# Autodesk Inventor assembly: Mechanism Platform
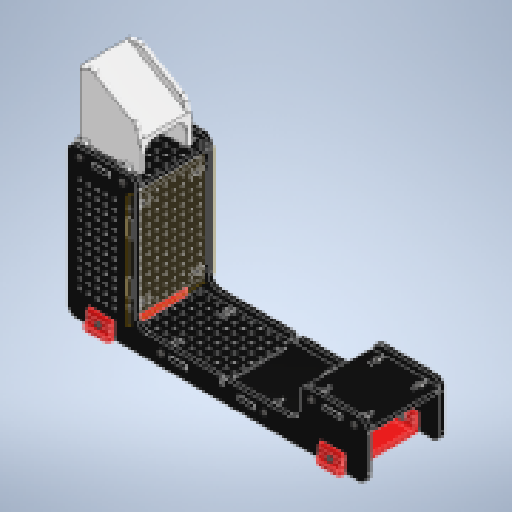
[picture p0: Inventor's stored thumbnail of the model, 512x512]
Saved by Autodesk Inventor 2025.1 (Build 291241000, 241)
## iProperties
Manager: Yassa Basem
Company: ENG 1P13
Created: 2024-06-07
Part Number: Mechanism Platform
Document SubType Name: Assembly
Designer: Alex Forbes
Checked By: Yassa Basem
Engineer: Alex Forbes
Author: A 1P13 IAI
Title: Mechanism Platform
## Documents named in this file (11)
- C:\Users\hanna\OneDrive - McMaster University\Documents\ENG 1P13A\Project 1\New folder (1)\Mechanism Platform.iam
- C:\Users\hanna\OneDrive - McMaster University\Documents\ENG 1P13A\Project 1\New folder (1)\Mounting Base Middle.ipt
- C:\Users\hanna\OneDrive - McMaster University\Documents\ENG 1P13A\Project 1\New folder (1)\Mounting Base Side.ipt
- C:\Users\hanna\OneDrive - McMaster University\Documents\ENG 1P13A\Project 1\New folder (1)\ANSI B 18.2.4.1 M - M4 x 0.7Style 1.ipt
- C:\Users\hanna\OneDrive - McMaster University\Documents\ENG 1P13A\Project 1\New folder (1)\Mounting Base Bottom.ipt
- C:\Users\hanna\OneDrive - McMaster University\Documents\ENG 1P13A\Project 1\New folder (1)\ANSI B18.6.7M - M4x0.7 x 20(4).ipt
- C:\Users\hanna\OneDrive - McMaster University\Documents\ENG 1P13A\Project 1\New folder (1)\Mounting Feet.ipt
- C:\Users\hanna\OneDrive - McMaster University\Documents\ENG 1P13A\Project 1\New folder (1)\Mounting Side Wall.ipt
- C:\Users\hanna\OneDrive - McMaster University\Documents\ENG 1P13A\Project 1\New folder (1)\Mounting Base Top.ipt
- C:\Users\hanna\OneDrive - McMaster University\Documents\ENG 1P13A\Project 1\New folder (1)\Top Ramp.ipt
- C:\Users\hanna\OneDrive - McMaster University\Documents\ENG 1P13A\Project 1\New folder (1)\M4 x 20mm Machine Screw.ipt
## Components (53 placed, 10 different names)
1. Top Ramp:1 — Insert:3, Insert:4, Insert:6, Insert:7, Insert:8, Insert:9, Insert:10, Insert:11, Angle:8, Angle:9, Angle:10, Angle:11
2. M4 x 20mm Machine Screw:1 — Insert:3, Angle:9
3. M4 x 20mm Machine Screw:2 — Insert:7, Angle:8
4. M4 x 20mm Machine Screw:3 — Insert:4, Angle:10
5. M4 x 20mm Machine Screw:4 — Insert:6, Angle:11
6. Mounting Side Wall:1 — Insert:1, Angle:1, Insert:2, Mate:1, Mate:2, Mate:3, Mate:4, Flush:1, Flush:2, Mate:5, Angle:3, Mate:6, Mate:7, Mate:8, Mate:9, Mate:50, Mate:51, Mate:52, Mate:53, Mate:109, Mate:110, Mate:111, Mate:129, Mate:130, Mate:131, Mate:133, Mate:134, Mate:135, Mate:145, Mate:146, Mate:147, Mate:149, Mate:150, Mate:151, Mate:157, Mate:158, Mate:159, Mate:169, Mate:170, Mate:171, Mate:173, Mate:174, Mate:175
7. Mounting Side Wall:2 — Mate:4, Flush:1, Flush:2, Mate:117, Mate:118, Mate:119, Mate:121, Mate:122, Mate:123, Mate:125, Mate:126, Mate:127, Mate:137, Mate:138, Mate:139, Mate:141, Mate:142, Mate:143, Mate:153, Mate:154, Mate:155, Mate:161, Mate:162, Mate:163, Mate:165, Mate:166, Mate:167
8. Mounting Base Top:1 — Mate:1, Mate:8, Mate:9, Mate:112, Mate:120, Mate:124, Mate:176, Angle:6, Angle:7, Insert:8, Insert:9, Insert:10, Insert:11
9. Mounting Base Middle:1 — Mate:2, Mate:52, Mate:53, Mate:144, Mate:148, Mate:152, Mate:156
10. Mounting Base Bottom:1 — Mate:3, Mate:50, Mate:51, Mate:160, Mate:164, Mate:168, Mate:172, Angle:4, Angle:5
11. Mounting Base Side:1 — Mate:5, Angle:3, Mate:6, Mate:7, Mate:128, Mate:132, Mate:136, Mate:140, Flush:3
12. Mounting Feet:1 — Insert:1, Angle:1, Angle:2, Mate:177, Mate:178, Mate:179, Mate:180, Mate:181, Mate:182, Mate:183, Mate:184
13. Mounting Feet:2 — Insert:2, Angle:2, Mate:185, Mate:186, Mate:187, Mate:188, Mate:189, Mate:190, Mate:191, Mate:192
14. Cross Recessed Pan Head Machine Screw - Type I - Metric M4x0.7 x 20:1 — Mate:173, Mate:174
15. Hex Nut Metric M4 x 0.7:1 — Mate:175, Mate:176
16. Cross Recessed Pan Head Machine Screw - Type I - Metric M4x0.7 x 20:7 — Mate:129, Mate:130
17. Hex Nut Metric M4 x 0.7:3 — Mate:131, Mate:132
18. Cross Recessed Pan Head Machine Screw - Type I - Metric M4x0.7 x 20:8 — Mate:133, Mate:134
19. Hex Nut Metric M4 x 0.7:5 — Mate:135, Mate:136
20. Cross Recessed Pan Head Machine Screw - Type I - Metric M4x0.7 x 20:5 — Mate:121, Mate:122
21. Hex Nut Metric M4 x 0.7:6 — Mate:123, Mate:124
22. Cross Recessed Pan Head Machine Screw - Type I - Metric M4x0.7 x 20:4 — Mate:117, Mate:118
23. Hex Nut Metric M4 x 0.7:7 — Mate:119, Mate:120
24. Cross Recessed Pan Head Machine Screw - Type I - Metric M4x0.7 x 20:6 — Mate:125, Mate:126
25. Hex Nut Metric M4 x 0.7:8 — Mate:127, Mate:128
26. Cross Recessed Pan Head Machine Screw - Type I - Metric M4x0.7 x 20:3 — Mate:137, Mate:138
27. Hex Nut Metric M4 x 0.7:10 — Mate:139, Mate:140
28. Cross Recessed Pan Head Machine Screw - Type I - Metric M4x0.7 x 20:10 — Mate:145, Mate:146
29. Hex Nut Metric M4 x 0.7:11 — Mate:147, Mate:148
30. Cross Recessed Pan Head Machine Screw - Type I - Metric M4x0.7 x 20:11 — Mate:149, Mate:150
31. Hex Nut Metric M4 x 0.7:13 — Mate:151, Mate:152
32. Cross Recessed Pan Head Machine Screw - Type I - Metric M4x0.7 x 20:9 — Mate:141, Mate:142
33. Hex Nut Metric M4 x 0.7:14 — Mate:143, Mate:144
34. Cross Recessed Pan Head Machine Screw - Type I - Metric M4x0.7 x 20:12 — Mate:153, Mate:154
35. Hex Nut Metric M4 x 0.7:16 — Mate:155, Mate:156
36. Cross Recessed Pan Head Machine Screw - Type I - Metric M4x0.7 x 20:13 — Mate:157, Mate:158
37. Hex Nut Metric M4 x 0.7:17 — Mate:159, Mate:160
38. Cross Recessed Pan Head Machine Screw - Type I - Metric M4x0.7 x 20:16 — Mate:169, Mate:170
39. Hex Nut Metric M4 x 0.7:18 — Mate:171, Mate:172
40. Cross Recessed Pan Head Machine Screw - Type I - Metric M4x0.7 x 20:14 — Mate:161, Mate:162
41. Hex Nut Metric M4 x 0.7:19 — Mate:163, Mate:164
42. Cross Recessed Pan Head Machine Screw - Type I - Metric M4x0.7 x 20:15 — Mate:165, Mate:166
43. Hex Nut Metric M4 x 0.7:20 — Mate:167, Mate:168
44. Cross Recessed Pan Head Machine Screw - Type I - Metric M4x0.7 x 20:2 — Mate:109, Mate:110
45. Hex Nut Metric M4 x 0.7:21 — Mate:111, Mate:112
46. Cross Recessed Pan Head Machine Screw - Type I - Metric M4x0.7 x 20:17 — Mate:177, Mate:178
47. Hex Nut Metric M4 x 0.7:22 — Mate:179, Mate:180, Angle:6
48. Cross Recessed Pan Head Machine Screw - Type I - Metric M4x0.7 x 20:18 — Mate:181, Mate:182
49. Hex Nut Metric M4 x 0.7:23 — Mate:183, Mate:184, Angle:7
50. Cross Recessed Pan Head Machine Screw - Type I - Metric M4x0.7 x 20:19 — Mate:185, Mate:186
51. Hex Nut Metric M4 x 0.7:24 — Mate:187, Mate:188, Angle:5
52. Cross Recessed Pan Head Machine Screw - Type I - Metric M4x0.7 x 20:20 — Mate:189, Mate:190
53. Hex Nut Metric M4 x 0.7:25 — Mate:191, Mate:192, Angle:4
## Relationships (117: Mate 93, Angle 11, Insert 10, Flush 3)
- Insert:1: Mounting Side Wall:1 ↔ Mounting Feet:1
- Angle:1 (0 deg): Mounting Side Wall:1 ↔ Mounting Feet:1
- Insert:2: Mounting Side Wall:1 ↔ Mounting Feet:2
- Angle:2 (0 deg): Mounting Feet:1 ↔ Mounting Feet:2
- Mate:1: Mounting Side Wall:1 ↔ Mounting Base Top:1
- Mate:2: Mounting Side Wall:1 ↔ Mounting Base Middle:1
- Mate:3: Mounting Side Wall:1 ↔ Mounting Base Bottom:1
- Mate:4 (102.3 mm): Mounting Side Wall:1 ↔ Mounting Side Wall:2
- Flush:1: Mounting Side Wall:1 ↔ Mounting Side Wall:2
- Flush:2: Mounting Side Wall:1 ↔ Mounting Side Wall:2
- Mate:5: Mounting Side Wall:1 ↔ Mounting Base Side:1
- Angle:3 (0 deg): Mounting Side Wall:1 ↔ Mounting Base Side:1
- Mate:6: Mounting Side Wall:1 ↔ Mounting Base Side:1
- Mate:7: Mounting Side Wall:1 ↔ Mounting Base Side:1
- Mate:8: Mounting Side Wall:1 ↔ Mounting Base Top:1
- Mate:9: Mounting Side Wall:1 ↔ Mounting Base Top:1
- Mate:50: Mounting Side Wall:1 ↔ Mounting Base Bottom:1
- Mate:51: Mounting Side Wall:1 ↔ Mounting Base Bottom:1
- Mate:52: Mounting Side Wall:1 ↔ Mounting Base Middle:1
- Mate:53: Mounting Side Wall:1 ↔ Mounting Base Middle:1
- Mate:109: Mounting Side Wall:1 ↔ Cross Recessed Pan Head Machine Screw - Type I - Metric M4x0.7 x 20:2
- Mate:110: Mounting Side Wall:1 ↔ Cross Recessed Pan Head Machine Screw - Type I - Metric M4x0.7 x 20:2
- Mate:111: Mounting Side Wall:1 ↔ Hex Nut Metric M4 x 0.7:21
- Mate:112: Mounting Base Top:1 ↔ Hex Nut Metric M4 x 0.7:21
- Mate:117: Mounting Side Wall:2 ↔ Cross Recessed Pan Head Machine Screw - Type I - Metric M4x0.7 x 20:4
- Mate:118: Mounting Side Wall:2 ↔ Cross Recessed Pan Head Machine Screw - Type I - Metric M4x0.7 x 20:4
- Mate:119: Mounting Side Wall:2 ↔ Hex Nut Metric M4 x 0.7:7
- Mate:120: Mounting Base Top:1 ↔ Hex Nut Metric M4 x 0.7:7
- Mate:121: Mounting Side Wall:2 ↔ Cross Recessed Pan Head Machine Screw - Type I - Metric M4x0.7 x 20:5
- Mate:122: Mounting Side Wall:2 ↔ Cross Recessed Pan Head Machine Screw - Type I - Metric M4x0.7 x 20:5
- Mate:123: Mounting Side Wall:2 ↔ Hex Nut Metric M4 x 0.7:6
- Mate:124: Mounting Base Top:1 ↔ Hex Nut Metric M4 x 0.7:6
- Mate:125: Mounting Side Wall:2 ↔ Cross Recessed Pan Head Machine Screw - Type I - Metric M4x0.7 x 20:6
- Mate:126: Mounting Side Wall:2 ↔ Cross Recessed Pan Head Machine Screw - Type I - Metric M4x0.7 x 20:6
- Mate:127: Mounting Side Wall:2 ↔ Hex Nut Metric M4 x 0.7:8
- Mate:128: Mounting Base Side:1 ↔ Hex Nut Metric M4 x 0.7:8
- Mate:129: Mounting Side Wall:1 ↔ Cross Recessed Pan Head Machine Screw - Type I - Metric M4x0.7 x 20:7
- Mate:130: Mounting Side Wall:1 ↔ Cross Recessed Pan Head Machine Screw - Type I - Metric M4x0.7 x 20:7
- Mate:131: Mounting Side Wall:1 ↔ Hex Nut Metric M4 x 0.7:3
- Mate:132: Mounting Base Side:1 ↔ Hex Nut Metric M4 x 0.7:3
- Mate:133: Mounting Side Wall:1 ↔ Cross Recessed Pan Head Machine Screw - Type I - Metric M4x0.7 x 20:8
- Mate:134: Mounting Side Wall:1 ↔ Cross Recessed Pan Head Machine Screw - Type I - Metric M4x0.7 x 20:8
- Mate:135: Mounting Side Wall:1 ↔ Hex Nut Metric M4 x 0.7:5
- Mate:136: Mounting Base Side:1 ↔ Hex Nut Metric M4 x 0.7:5
- Mate:137: Mounting Side Wall:2 ↔ Cross Recessed Pan Head Machine Screw - Type I - Metric M4x0.7 x 20:3
- Mate:138: Mounting Side Wall:2 ↔ Cross Recessed Pan Head Machine Screw - Type I - Metric M4x0.7 x 20:3
- Mate:139: Mounting Side Wall:2 ↔ Hex Nut Metric M4 x 0.7:10
- Mate:140: Mounting Base Side:1 ↔ Hex Nut Metric M4 x 0.7:10
- Mate:141: Mounting Side Wall:2 ↔ Cross Recessed Pan Head Machine Screw - Type I - Metric M4x0.7 x 20:9
- Mate:142: Mounting Side Wall:2 ↔ Cross Recessed Pan Head Machine Screw - Type I - Metric M4x0.7 x 20:9
- Mate:143: Mounting Side Wall:2 ↔ Hex Nut Metric M4 x 0.7:14
- Mate:144: Mounting Base Middle:1 ↔ Hex Nut Metric M4 x 0.7:14
- Mate:145: Mounting Side Wall:1 ↔ Cross Recessed Pan Head Machine Screw - Type I - Metric M4x0.7 x 20:10
- Mate:146: Mounting Side Wall:1 ↔ Cross Recessed Pan Head Machine Screw - Type I - Metric M4x0.7 x 20:10
- Mate:147: Mounting Side Wall:1 ↔ Hex Nut Metric M4 x 0.7:11
- Mate:148: Mounting Base Middle:1 ↔ Hex Nut Metric M4 x 0.7:11
- Mate:149: Mounting Side Wall:1 ↔ Cross Recessed Pan Head Machine Screw - Type I - Metric M4x0.7 x 20:11
- Mate:150: Mounting Side Wall:1 ↔ Cross Recessed Pan Head Machine Screw - Type I - Metric M4x0.7 x 20:11
- Mate:151: Mounting Side Wall:1 ↔ Hex Nut Metric M4 x 0.7:13
- Mate:152: Mounting Base Middle:1 ↔ Hex Nut Metric M4 x 0.7:13
- Mate:153: Mounting Side Wall:2 ↔ Cross Recessed Pan Head Machine Screw - Type I - Metric M4x0.7 x 20:12
- Mate:154: Mounting Side Wall:2 ↔ Cross Recessed Pan Head Machine Screw - Type I - Metric M4x0.7 x 20:12
- Mate:155: Mounting Side Wall:2 ↔ Hex Nut Metric M4 x 0.7:16
- Mate:156: Mounting Base Middle:1 ↔ Hex Nut Metric M4 x 0.7:16
- Mate:157: Mounting Side Wall:1 ↔ Cross Recessed Pan Head Machine Screw - Type I - Metric M4x0.7 x 20:13
- Mate:158: Mounting Side Wall:1 ↔ Cross Recessed Pan Head Machine Screw - Type I - Metric M4x0.7 x 20:13
- Mate:159: Mounting Side Wall:1 ↔ Hex Nut Metric M4 x 0.7:17
- Mate:160: Mounting Base Bottom:1 ↔ Hex Nut Metric M4 x 0.7:17
- Mate:161: Mounting Side Wall:2 ↔ Cross Recessed Pan Head Machine Screw - Type I - Metric M4x0.7 x 20:14
- Mate:162: Mounting Side Wall:2 ↔ Cross Recessed Pan Head Machine Screw - Type I - Metric M4x0.7 x 20:14
- Mate:163: Mounting Side Wall:2 ↔ Hex Nut Metric M4 x 0.7:19
- Mate:164: Mounting Base Bottom:1 ↔ Hex Nut Metric M4 x 0.7:19
- Mate:165: Mounting Side Wall:2 ↔ Cross Recessed Pan Head Machine Screw - Type I - Metric M4x0.7 x 20:15
- Mate:166: Mounting Side Wall:2 ↔ Cross Recessed Pan Head Machine Screw - Type I - Metric M4x0.7 x 20:15
- Mate:167: Mounting Side Wall:2 ↔ Hex Nut Metric M4 x 0.7:20
- Mate:168: Mounting Base Bottom:1 ↔ Hex Nut Metric M4 x 0.7:20
- Mate:169: Mounting Side Wall:1 ↔ Cross Recessed Pan Head Machine Screw - Type I - Metric M4x0.7 x 20:16
- Mate:170: Mounting Side Wall:1 ↔ Cross Recessed Pan Head Machine Screw - Type I - Metric M4x0.7 x 20:16
- Mate:171: Mounting Side Wall:1 ↔ Hex Nut Metric M4 x 0.7:18
- Mate:172: Mounting Base Bottom:1 ↔ Hex Nut Metric M4 x 0.7:18
- Mate:173: Mounting Side Wall:1 ↔ Cross Recessed Pan Head Machine Screw - Type I - Metric M4x0.7 x 20:1
- Mate:174: Mounting Side Wall:1 ↔ Cross Recessed Pan Head Machine Screw - Type I - Metric M4x0.7 x 20:1
- Mate:175: Mounting Side Wall:1 ↔ Hex Nut Metric M4 x 0.7:1
- Mate:176: Mounting Base Top:1 ↔ Hex Nut Metric M4 x 0.7:1
- Mate:177: Mounting Feet:1 ↔ Cross Recessed Pan Head Machine Screw - Type I - Metric M4x0.7 x 20:17
- Mate:178: Mounting Feet:1 ↔ Cross Recessed Pan Head Machine Screw - Type I - Metric M4x0.7 x 20:17
- Mate:179: Mounting Feet:1 ↔ Hex Nut Metric M4 x 0.7:22
- Mate:180: Mounting Feet:1 ↔ Hex Nut Metric M4 x 0.7:22
- Mate:181: Mounting Feet:1 ↔ Cross Recessed Pan Head Machine Screw - Type I - Metric M4x0.7 x 20:18
- Mate:182: Mounting Feet:1 ↔ Cross Recessed Pan Head Machine Screw - Type I - Metric M4x0.7 x 20:18
- Mate:183: Mounting Feet:1 ↔ Hex Nut Metric M4 x 0.7:23
- Mate:184: Mounting Feet:1 ↔ Hex Nut Metric M4 x 0.7:23
- Mate:185: Mounting Feet:2 ↔ Cross Recessed Pan Head Machine Screw - Type I - Metric M4x0.7 x 20:19
- Mate:186: Mounting Feet:2 ↔ Cross Recessed Pan Head Machine Screw - Type I - Metric M4x0.7 x 20:19
- Mate:187: Mounting Feet:2 ↔ Hex Nut Metric M4 x 0.7:24
- Mate:188: Mounting Feet:2 ↔ Hex Nut Metric M4 x 0.7:24
- Mate:189: Mounting Feet:2 ↔ Cross Recessed Pan Head Machine Screw - Type I - Metric M4x0.7 x 20:20
- Mate:190: Mounting Feet:2 ↔ Cross Recessed Pan Head Machine Screw - Type I - Metric M4x0.7 x 20:20
- Mate:191: Mounting Feet:2 ↔ Hex Nut Metric M4 x 0.7:25
- Mate:192: Mounting Feet:2 ↔ Hex Nut Metric M4 x 0.7:25
- Angle:4 (0 deg): Mounting Base Bottom:1 ↔ Hex Nut Metric M4 x 0.7:25
- Angle:5 (0 deg): Mounting Base Bottom:1 ↔ Hex Nut Metric M4 x 0.7:24
- Angle:6 (0 deg): Mounting Base Top:1 ↔ Hex Nut Metric M4 x 0.7:22
- Angle:7 (0 deg): Mounting Base Top:1 ↔ Hex Nut Metric M4 x 0.7:23
- Insert:3: Top Ramp:1 ↔ M4 x 20mm Machine Screw:1
- Insert:4: Top Ramp:1 ↔ M4 x 20mm Machine Screw:3
- Insert:6: Top Ramp:1 ↔ M4 x 20mm Machine Screw:4
- Insert:7: Top Ramp:1 ↔ M4 x 20mm Machine Screw:2
- Insert:8: Top Ramp:1 ↔ Mounting Base Top:1
- Insert:9: Top Ramp:1 ↔ Mounting Base Top:1
- Insert:10: Top Ramp:1 ↔ Mounting Base Top:1
- Insert:11: Top Ramp:1 ↔ Mounting Base Top:1
- Angle:8 (0 deg): Top Ramp:1 ↔ M4 x 20mm Machine Screw:2
- Angle:9 (0 deg): Top Ramp:1 ↔ M4 x 20mm Machine Screw:1
- Angle:10 (0 deg): Top Ramp:1 ↔ M4 x 20mm Machine Screw:3
- Angle:11 (0 deg): Top Ramp:1 ↔ M4 x 20mm Machine Screw:4
- Flush:3: Mounting Base Side:1
